# Autodesk Inventor assembly: Linear-Rail MGN12H
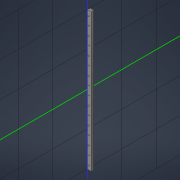
[picture p0: Inventor's stored thumbnail of the model, 180x180]
Saved by Autodesk Inventor 2022.2 (Build 262287010, 287A)
## iProperties
Created: 2022-03-15
Part Number: Linear-Rail MGN12H
Document SubType Name: Assembly
Designer: sleib
Author: sleib
## Documents named in this file (3)
- C:\Users\sleib\Projekte\Voron-2\CAD\Inventor\Linear-Rail MGN12H.iam
- C:\Users\sleib\Projekte\Voron-2\CAD\Inventor\MGN12H Linear-Rail (400mm).ipt
- C:\Users\sleib\Projekte\Voron-2\CAD\Inventor\M3x8 SHCS.ipt
## Components (9 placed, 2 different names)
1. MGN12H Linear-Rail (400mm):1 — Passend:1, Passend:2, Passend:3, Passend:4, Passend:5, Passend:6, Passend:7, Passend:8, Passend:9, Passend:10, Passend:11, Passend:12, Passend:13, Passend:14, Passend:15, Passend:16
2. M3x8 SHCS:1 — Passend:1, Passend:16
3. M3x8 SHCS:2 — Passend:2, Passend:15
4. M3x8 SHCS:3 — Passend:3, Passend:14
5. M3x8 SHCS:4 — Passend:4, Passend:13
6. M3x8 SHCS:5 — Passend:8, Passend:9
7. M3x8 SHCS:6 — Passend:7, Passend:10
8. M3x8 SHCS:7 — Passend:6, Passend:11
9. M3x8 SHCS:8 — Passend:5, Passend:12
## Relationships (16: Mate 16)
- Passend:1 [Mate]: MGN12H Linear-Rail (400mm):1 ↔ M3x8 SHCS:1
- Passend:2 [Mate]: MGN12H Linear-Rail (400mm):1 ↔ M3x8 SHCS:2
- Passend:3 [Mate]: MGN12H Linear-Rail (400mm):1 ↔ M3x8 SHCS:3
- Passend:4 [Mate]: MGN12H Linear-Rail (400mm):1 ↔ M3x8 SHCS:4
- Passend:5 [Mate]: MGN12H Linear-Rail (400mm):1 ↔ M3x8 SHCS:8
- Passend:6 [Mate]: MGN12H Linear-Rail (400mm):1 ↔ M3x8 SHCS:7
- Passend:7 [Mate]: MGN12H Linear-Rail (400mm):1 ↔ M3x8 SHCS:6
- Passend:8 [Mate]: MGN12H Linear-Rail (400mm):1 ↔ M3x8 SHCS:5
- Passend:9 [Mate]: MGN12H Linear-Rail (400mm):1 ↔ M3x8 SHCS:5
- Passend:10 [Mate]: MGN12H Linear-Rail (400mm):1 ↔ M3x8 SHCS:6
- Passend:11 [Mate]: MGN12H Linear-Rail (400mm):1 ↔ M3x8 SHCS:7
- Passend:12 [Mate]: MGN12H Linear-Rail (400mm):1 ↔ M3x8 SHCS:8
- Passend:13 [Mate]: MGN12H Linear-Rail (400mm):1 ↔ M3x8 SHCS:4
- Passend:14 [Mate]: MGN12H Linear-Rail (400mm):1 ↔ M3x8 SHCS:3
- Passend:15 [Mate]: MGN12H Linear-Rail (400mm):1 ↔ M3x8 SHCS:2
- Passend:16 [Mate]: MGN12H Linear-Rail (400mm):1 ↔ M3x8 SHCS:1
